# Autodesk Inventor assembly: Leg_Loadpipe_Mount_MIR
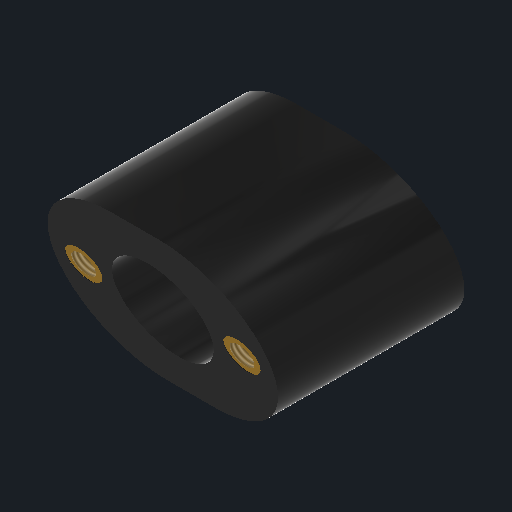
[picture p0: Inventor's stored thumbnail of the model, 512x512]
Saved by Autodesk Inventor 2024.1 (Build 281209000, 209)
## iProperties
Created: 2023-06-09
Part Number: Leg_Loadpipe_Mount_MIR
Document SubType Name: Assembly
Designer: dzw04
Author: dzw04
## Documents named in this file (4)
- C:\Users\dzw04\Saxion\Mechatronica Lectoraat LMECH LED - Database ARG\Component_Database\SARAX\01. CAD\01. 3D_Drawing\02. Sub_Assemblies\Landing_Gear\02. Sub_Assemblies\Leg_Loadpipe_Mount_MIR.iam
- C:\Users\dzw04\Saxion\Mechatronica Lectoraat LMECH LED - Database ARG\Component_Database\SARAX\01. CAD\01. 3D_Drawing\02. Sub_Assemblies\Landing_Gear\01. Parts\Leg_Loadpipe_Mount_MIR.ipt
- C:\Users\dzw04\Saxion\Mechatronica Lectoraat LMECH LED - Database ARG\Component_Database\SARAX\01. CAD\01. 3D_Drawing\01. Parts\Threaded_Insert_M3x4_MIR.ipt
- C:\Users\dzw04\OneDrive - Saxion\Documenten\Inventor\Content Center Files\R2024\en-US\DIN 913\DIN 913 - M4 x 4.ipt
## Components (7 placed, 3 different names)
1. Leg_Loadpipe_Mount_MIR:1 — Mate:5, Flush:1, Mate:4, Flush:2, Mate:3, Flush:3, Mate:1, Flush:5, Mate:2, Flush:4, Mate:6
2. Threaded_Insert_M3x4_MIR:1 — Mate:5, Flush:1
3. Threaded_Insert_M3x4_MIR:2 — Mate:4, Flush:2
4. Threaded_Insert_M3x4_MIR:3 — Mate:3, Flush:3
5. Threaded_Insert_M3x4_MIR:4 — Mate:1, Flush:5
6. Threaded_Insert_M3x4_MIR:5 — Mate:2, Flush:4
7. DIN 913 M4 x 4:1 — Mate:6
## Relationships (11: Mate 6, Flush 5)
- Mate:5: Leg_Loadpipe_Mount_MIR:1 ↔ Threaded_Insert_M3x4_MIR:1
- Flush:1: Leg_Loadpipe_Mount_MIR:1 ↔ Threaded_Insert_M3x4_MIR:1
- Mate:4: Leg_Loadpipe_Mount_MIR:1 ↔ Threaded_Insert_M3x4_MIR:2
- Flush:2: Leg_Loadpipe_Mount_MIR:1 ↔ Threaded_Insert_M3x4_MIR:2
- Mate:3: Leg_Loadpipe_Mount_MIR:1 ↔ Threaded_Insert_M3x4_MIR:3
- Flush:3: Leg_Loadpipe_Mount_MIR:1 ↔ Threaded_Insert_M3x4_MIR:3
- Mate:1: Leg_Loadpipe_Mount_MIR:1 ↔ Threaded_Insert_M3x4_MIR:4
- Flush:5: Leg_Loadpipe_Mount_MIR:1 ↔ Threaded_Insert_M3x4_MIR:4
- Mate:2: Leg_Loadpipe_Mount_MIR:1 ↔ Threaded_Insert_M3x4_MIR:5
- Flush:4: Leg_Loadpipe_Mount_MIR:1 ↔ Threaded_Insert_M3x4_MIR:5
- Mate:6: Leg_Loadpipe_Mount_MIR:1 ↔ DIN 913 M4 x 4:1
